# Autodesk Inventor assembly: sort support V2
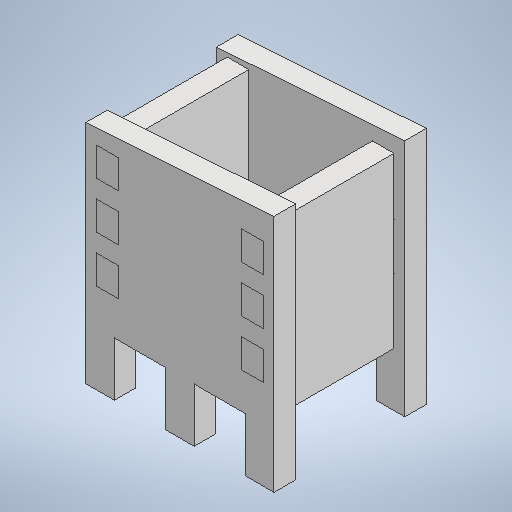
[picture p0: Inventor's stored thumbnail of the model, 512x512]
Saved by Autodesk Inventor 2025.3 (Build 293356000, 356)
## iProperties
Created: 2026-04-30
Part Number: sort support V2
Document SubType Name: Assembly
Designer: kamal
Author: kamal
## Documents named in this file (3)
- C:\Users\kamal\OneDrive\Desktop\Personal\semester 4\Basics of Mechatronics\Full Assembly\sort support V2.iam
- C:\Users\kamal\OneDrive\Desktop\Personal\semester 4\Basics of Mechatronics\Full Assembly\sort support V2 wall 1.ipt
- C:\Users\kamal\OneDrive\Desktop\Personal\semester 4\Basics of Mechatronics\Full Assembly\sort support V2 wall 2.ipt
## Components (4 placed, 2 different names)
1. sort support V2 wall 1:1 — Mate:1, Mate:2, Mate:3, Mate:4, Mate:5
2. sort support V2 wall 2:1 — Mate:1, Mate:2, Mate:6, Mate:7
3. sort support V2 wall 2:2 — Mate:3, Mate:4, Mate:5
4. sort support V2 wall 1:2 — Mate:6, Mate:7
## Relationships (7: Mate 7)
- Mate:1: sort support V2 wall 1:1 ↔ sort support V2 wall 2:1
- Mate:2: sort support V2 wall 1:1 ↔ sort support V2 wall 2:1
- Mate:3: sort support V2 wall 1:1 ↔ sort support V2 wall 2:2
- Mate:4: sort support V2 wall 1:1 ↔ sort support V2 wall 2:2
- Mate:5: sort support V2 wall 1:1 ↔ sort support V2 wall 2:2
- Mate:6: sort support V2 wall 2:1 ↔ sort support V2 wall 1:2
- Mate:7: sort support V2 wall 2:1 ↔ sort support V2 wall 1:2
